# Autodesk Inventor assembly: CyclV2
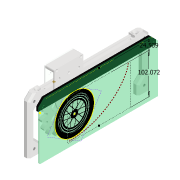
[picture p0: Inventor's stored thumbnail of the model, 180x180]
Saved by Autodesk Inventor 2020 (Build 240168000, 168)
## iProperties
Created: 2021-07-09
Part Number: CyclV2
Document SubType Name: Assembly
Designer: Aidan Lee
Author: Aidan Lee
## Documents named in this file (11)
- C:\Users\hobly\Dropbox\Aidan Lee\Mechanics_Walk\Brachistochrone-v2\CycloidDrawer.iam
- C:\Users\hobly\Dropbox\Aidan Lee\Mechanics_Walk\Brachistochrone-v2\BR-11-racktop.ipt
- C:\Users\hobly\Dropbox\Aidan Lee\Mechanics_Walk\Brachistochrone-v2\BR-12-rackbottom.ipt
- C:\Users\hobly\Dropbox\Aidan Lee\Mechanics_Walk\Brachistochrone-v2\BR-14-trolleyside.ipt
- C:\Users\hobly\Dropbox\Aidan Lee\Mechanics_Walk\Brachistochrone-v2\BR-13-trolleycentre.ipt
- C:\Users\hobly\Dropbox\Aidan Lee\Mechanics_Walk\Brachistochrone-v2\BR-15-pinion.ipt
- C:\Users\hobly\Dropbox\Aidan Lee\Mechanics_Walk\Brachistochrone-v2\BR-16-wheel.ipt
- C:\Users\hobly\Dropbox\Aidan Lee\Mechanics_Walk\Brachistochrone-v2\BR-17-road.ipt
- C:\Users\hobly\Dropbox\Aidan Lee\Mechanics_Walk\Brachistochrone-v2\BR-18-glass.ipt
- C:\Users\hobly\Dropbox\Aidan Lee\Mechanics_Walk\Brachistochrone-v2\BR-19-rackstandright.ipt
- C:\Users\hobly\Dropbox\Aidan Lee\Mechanics_Walk\Brachistochrone-v2\BR-20-rackstandleft.ipt
## Components (11 placed, 10 different names)
1. BR-11-racktop:1 — Mate:5, Mate:15, Mate:16, Mate:21, Flush:4, Mate:25, Mate:28
2. BR-12-rackbottom:1 — Mate:5, Mate:21, Flush:4, Mate:24, Mate:29
3. BR-13-trolleycentre:1 — Mate:9, Mate:10, Mate:11, Mate:12, Mate:15
4. BR-14-trolleyside:2 — Mate:9, Mate:10, Mate:13, Mate:16, Mate:17
5. BR-14-trolleyside:3 — Mate:11, Mate:12, Mate:19
6. BR-15-pinion:1 — Mate:13, Mate:17, Mate:20, Flush:3
7. BR-16-wheel:1 — Mate:19, Mate:20, Flush:3
8. BR-17-road:1 — Mate:30, Mate:31, Mate:32, Mate:33, Mate:34, Flush:6
9. BR-18-glass:1 — Mate:33, Mate:34, Flush:6
10. BR-19-rackstandright:1 — Mate:24, Mate:25, Mate:32
11. BR-20-rackstandleft:1 — Flush:5, Mate:26, Mate:27, Mate:28, Mate:29, Mate:30, Mate:31
## Relationships (27: Mate 23, Flush 4)
- Mate:5: BR-11-racktop:1 ↔ BR-12-rackbottom:1
- Mate:9: BR-13-trolleycentre:1 ↔ BR-14-trolleyside:2
- Mate:10: BR-13-trolleycentre:1 ↔ BR-14-trolleyside:2
- Mate:11: BR-13-trolleycentre:1 ↔ BR-14-trolleyside:3
- Mate:12: BR-13-trolleycentre:1 ↔ BR-14-trolleyside:3
- Mate:13: BR-14-trolleyside:2 ↔ BR-15-pinion:1
- Mate:15 (28.5 mm): BR-11-racktop:1 ↔ BR-13-trolleycentre:1
- Mate:16 (2 mm): BR-11-racktop:1 ↔ BR-14-trolleyside:2
- Mate:17 (2 mm): BR-14-trolleyside:2 ↔ BR-15-pinion:1
- Mate:19 (4 mm): BR-14-trolleyside:3 ↔ BR-16-wheel:1
- Mate:20: BR-15-pinion:1 ↔ BR-16-wheel:1
- Flush:3: BR-15-pinion:1 ↔ BR-16-wheel:1
- Mate:21: BR-11-racktop:1 ↔ BR-12-rackbottom:1
- Flush:4: BR-11-racktop:1 ↔ BR-12-rackbottom:1
- Mate:24: BR-12-rackbottom:1 ↔ BR-19-rackstandright:1
- Mate:25: BR-11-racktop:1 ↔ BR-19-rackstandright:1
- Flush:5: BR-20-rackstandleft:1
- Mate:26: BR-20-rackstandleft:1
- Mate:27: BR-20-rackstandleft:1
- Mate:28: BR-11-racktop:1 ↔ BR-20-rackstandleft:1
- Mate:29: BR-12-rackbottom:1 ↔ BR-20-rackstandleft:1
- Mate:30: BR-17-road:1 ↔ BR-20-rackstandleft:1
- Mate:31 (15 mm): BR-17-road:1 ↔ BR-20-rackstandleft:1
- Mate:32: BR-17-road:1 ↔ BR-19-rackstandright:1
- Mate:33: BR-17-road:1 ↔ BR-18-glass:1
- Mate:34: BR-17-road:1 ↔ BR-18-glass:1
- Flush:6: BR-17-road:1 ↔ BR-18-glass:1
